# Autodesk Inventor assembly: Hand
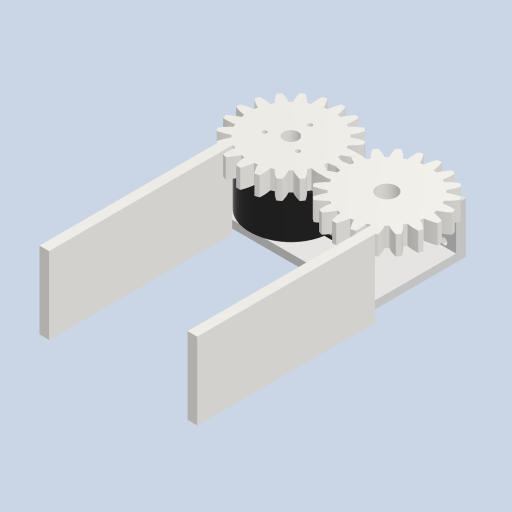
[picture p0: Inventor's stored thumbnail of the model, 512x512]
Saved by Autodesk Inventor 2023 (Build 270158000, 158)
## iProperties
Created: 2024-11-08
Part Number: Hand
Document SubType Name: Assembly
Designer: kiyo
Author: kiyo
## Documents named in this file (7)
- D:\GitHub\inventor\syu-si\OfficeRobot\Manipulator\Hand.iam
- D:\GitHub\inventor\syu-si\OfficeRobot\Manipulator\hand-gearbox.ipt
- D:\GitHub\inventor\syu-si\OfficeRobot\Manipulator\hand-nail-1.ipt
- D:\GitHub\inventor\syu-si\OfficeRobot\Manipulator\hand-nail-2.ipt
- D:\GitHub\inventor\syu-si\OfficeRobot\ReadyMade\Steadywin\GIM3505-8.ipt
- D:\GitHub\inventor\syu-si\OfficeRobot\ReadyMade\Screw\D3040-7130B.ipt
- D:\GitHub\inventor\syu-si\OfficeRobot\ReadyMade\Screw\D4050-9120B.ipt
## Components (6 placed, 6 different names)
1. hand-gearbox:1 — 挿入:3, 挿入:4, 挿入:5
2. 平歯車1:1 — 挿入:6
3. 平歯車2:1 — 挿入:2
4. GIM3505-8:1 — 挿入:4, 挿入:5, 挿入:6
5. D3040-7130B:1 — 挿入:1, 挿入:3
6. D4050-9120B:1 — 挿入:1, 挿入:2
## Relationships (6: Insert 6)
- 挿入:1 [Insert]: D3040-7130B:1 ↔ D4050-9120B:1
- 挿入:2 [Insert]: 平歯車2:1 ↔ D4050-9120B:1
- 挿入:3 [Insert]: hand-gearbox:1 ↔ D3040-7130B:1
- 挿入:4 [Insert]: hand-gearbox:1 ↔ GIM3505-8:1
- 挿入:5 [Insert]: hand-gearbox:1 ↔ GIM3505-8:1
- 挿入:6 [Insert]: 平歯車1:1 ↔ GIM3505-8:1
